# Autodesk Inventor assembly: Legstretcher_MIR
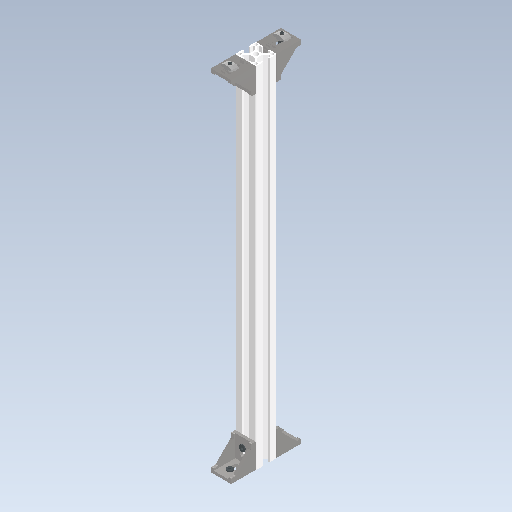
[picture p0: Inventor's stored thumbnail of the model, 512x512]
Saved by Autodesk Inventor 2020.2 (Build 242310000, 310)
## iProperties
Created: 2020-07-25
Part Number: Legstretcher_MIR
Document SubType Name: Assembly
Designer: JK
Author: JK
## Documents named in this file (3)
- C:\Users\JK\Documents\Inventor\Mesa\Legstretcher_MIR.iam
- C:\Users\JK\Documents\Inventor\Mesa\30x30x500_MIR.ipt
- C:\Users\JK\Documents\Inventor\Mesa\Cornerassembly_MIR.iam
## Components (5 placed, 2 different names)
1. 30x30x500_MIR:1 — Flush:2, Flush:1, Mate:1, Flush:6, Flush:5, Mate:3, Flush:3, Mate:2, Flush:8, Flush:7, Mate:4
2. Cornerassembly_MIR:1 [sub-assembly] — Flush:2, Flush:1, Mate:1, Flush:4
3. Cornerassembly_MIR:2 [sub-assembly] — Flush:6, Flush:5, Mate:3
4. Cornerassembly_MIR:3 [sub-assembly] — Flush:4, Flush:3, Mate:2
5. Cornerassembly_MIR:4 [sub-assembly] — Flush:8, Flush:7, Mate:4
## Relationships (12: Flush 8, Mate 4)
- Flush:2 (0.5 mm): 30x30x500_MIR:1 ↔ Cornerassembly_MIR:1
- Flush:1: 30x30x500_MIR:1 ↔ Cornerassembly_MIR:1
- Mate:1: 30x30x500_MIR:1 ↔ Cornerassembly_MIR:1
- Flush:6: 30x30x500_MIR:1 ↔ Cornerassembly_MIR:2
- Flush:5 (0.5 mm): 30x30x500_MIR:1 ↔ Cornerassembly_MIR:2
- Mate:3: 30x30x500_MIR:1 ↔ Cornerassembly_MIR:2
- Flush:4: Cornerassembly_MIR:1 ↔ Cornerassembly_MIR:3
- Flush:3 (0.5 mm): 30x30x500_MIR:1 ↔ Cornerassembly_MIR:3
- Mate:2: 30x30x500_MIR:1 ↔ Cornerassembly_MIR:3
- Flush:8: 30x30x500_MIR:1 ↔ Cornerassembly_MIR:4
- Flush:7 (0.5 mm): 30x30x500_MIR:1 ↔ Cornerassembly_MIR:4
- Mate:4: 30x30x500_MIR:1 ↔ Cornerassembly_MIR:4
